# Autodesk Inventor assembly: MG-Dribblingwelle v2
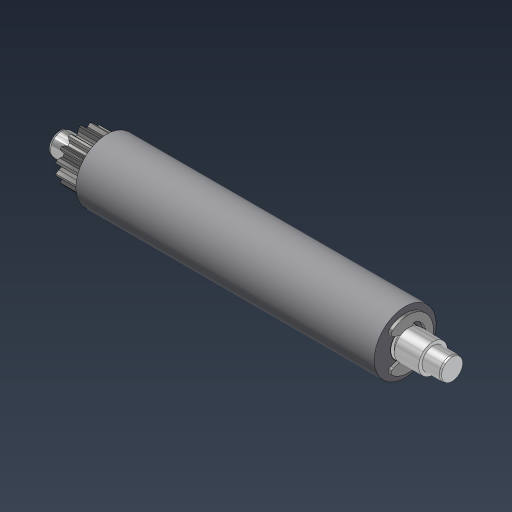
[picture p0: Inventor's stored thumbnail of the model, 512x512]
Saved by Autodesk Inventor 2023.1 (Build 271208000, 208)
## iProperties
Part Number: MG-Dribblingwelle v2
Material: Generisch
Document SubType Name: Assembly
Designer: rYan
Mass: 14.5523 g
Surface Area: 62.9337 cm^2
Volume: 6.77072 cm^3
Author: rYan
## Documents named in this file (5)
- D:\TIGERsGIT\Hardware\mechanik\2024\Inventor\Robot\Dribbler\MG-Dribblingwelle v2.iam
- D:\TIGERsGIT\Hardware\mechanik\2024\Inventor\Robot\Dribbler\Dribblingwelle.ipt
- D:\TIGERsGIT\Hardware\mechanik\2024\Inventor\Inhaltscenter\de-DE\DIN 6799\DIN 6799 - 5 6.ipt
- D:\TIGERsGIT\Hardware\mechanik\2024\Inventor\Purchased Parts\Zahnrad z14 Modul 0.7 Schnecke.ipt
- D:\TIGERsGIT\Hardware\mechanik\2024\Inventor\Robot\Dribbler\Dribblerschnecke v4.ipt
## Components (4 placed, 4 different names)
1. Dribblingwelle:1 — Einfügen:6, Fluchtend:2, Fluchtend:3, Fluchtend:4, Passend:4, Fluchtend:5, Einfügen:7
2. DIN 6799 5:2 — Einfügen:6
3. Dribblerschnecke v4:1 — Passend:4, Fluchtend:5
4. Zahnrad z14 Modul 0.7 Schnecke:1 — Einfügen:7
## Relationships (7: Flush 4, Insert 2, Mate 1)
- Einfügen:6 [Insert]: Dribblingwelle:1 ↔ DIN 6799 5:2
- Fluchtend:2 [Flush]: Dribblingwelle:1
- Fluchtend:3 [Flush]: Dribblingwelle:1
- Fluchtend:4 [Flush]: Dribblingwelle:1
- Passend:4 [Mate]: Dribblingwelle:1 ↔ Dribblerschnecke v4:1
- Fluchtend:5 [Flush]: Dribblingwelle:1 ↔ Dribblerschnecke v4:1
- Einfügen:7 [Insert]: Dribblingwelle:1 ↔ Zahnrad z14 Modul 0.7 Schnecke:1
